# Autodesk Inventor assembly: Assembly1
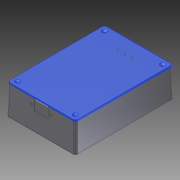
[picture p0: Inventor's stored thumbnail of the model, 180x180]
Saved by Autodesk Inventor 2012 (Build 160160000, 160)
## iProperties
Created: 2017-06-15
Part Number: Assembly1
Document SubType Name: Assembly
Designer: Brandon
Author: Brandon
## Documents named in this file (6)
- C:\Users\Brandon\Dropbox\Admiral Instruments Dropbox\power supply\power supply enclosure\Assembly1.iam
- C:\Users\Brandon\Dropbox\Admiral Instruments Dropbox\power supply\power supply enclosure\AC entry module.ipt
- C:\Users\Brandon\Dropbox\Admiral Instruments Dropbox\power supply\power supply enclosure\Bud enclosure CU389.ipt
- C:\Users\Brandon\Dropbox\Admiral Instruments Dropbox\power supply\power supply enclosure\power supply pcb.ipt
- C:\Users\Brandon\Dropbox\Admiral Instruments Dropbox\Squidstat Plus 2.0 (single channel, with EIS)\Enclosure\DB9 connector 2017_06_14.ipt
- C:\Users\Brandon\Dropbox\Admiral Instruments Dropbox\power supply\power supply enclosure\lid.ipt
## Components (5 placed, 5 different names)
1. AC entry module:1 — Insert:2, Angle:2
2. Bud enclosure CU389:1 — Insert:1, Angle:1, Flush:1
3. power supply pcb:1 — Insert:1, Angle:1, Insert:2, Angle:2, Insert:3, Angle:3
4. DB9 connector 2017_06_14:1 — Insert:3, Angle:3
5. lid:1 — Flush:1
## Relationships (7: Insert 3, Angle 3, Flush 1)
- Insert:1 (28.3464 mm): Bud enclosure CU389:1 ↔ power supply pcb:1
- Angle:1 (0 deg): Bud enclosure CU389:1 ↔ power supply pcb:1
- Insert:2: AC entry module:1 ↔ power supply pcb:1
- Angle:2 (0 deg): AC entry module:1 ↔ power supply pcb:1
- Insert:3: power supply pcb:1 ↔ DB9 connector 2017_06_14:1
- Angle:3 (0 deg): power supply pcb:1 ↔ DB9 connector 2017_06_14:1
- Flush:1: Bud enclosure CU389:1 ↔ lid:1
